# Autodesk Inventor assembly: Pancake Pneumatic Cylinder (217-2778)
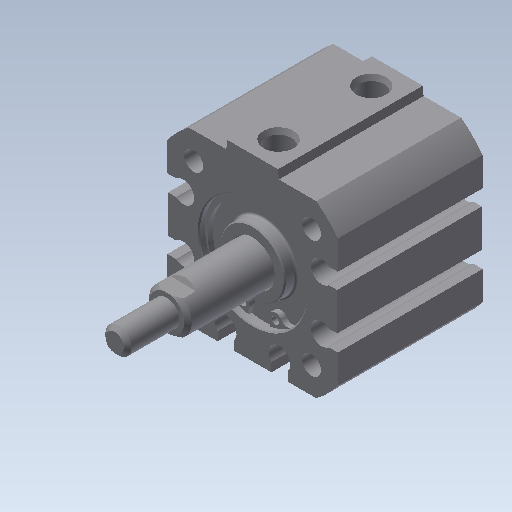
[picture p0: Inventor's stored thumbnail of the model, 512x512]
Saved by Autodesk Inventor 2020 (Build 240168000, 168)
## iProperties
Created: 2014-08-06
Part Number: Pancake Pneumatic Cylinder (217-2778)
Description: STEP AP203
Document SubType Name: Assembly
Designer: mavericks
Sending System: SolidWorks 2014
Preprocessor: SwSTEP 2.0
Title: 217-2778-001 Rev2.STEP
Revision Number: ANY
## Documents named in this file (4)
- T:\EIT\2022 Rapid React\COMMON PARTS\AIR CYLINDERS\Pancake cylinders\Pancake Pneumatic Cylinder (217-2778).iam
- T:\EIT\2022 Rapid React\COMMON PARTS\AIR CYLINDERS\Pancake cylinders\217-2778-NCQ8A075-050M_NCQ8 Tube_075A.ipt
- T:\EIT\2022 Rapid React\COMMON PARTS\AIR CYLINDERS\Pancake cylinders\217-2778-NCQ8A075-050M_NCQ8 Rod_075M.ipt
- T:\EIT\2022 Rapid React\COMMON PARTS\AIR CYLINDERS\Pancake cylinders\217-2778-NCQ8A075-050M_Snap Ring_075.ipt
## Components (3 placed, 3 different names)
1. 217-2778-NCQ8A075-050M_NCQ8 Tube_075A_1 — Mate:1, Mate:2
2. 217-2778-NCQ8A075-050M_NCQ8 Rod_075M_2 — Mate:1, Mate:2
3. 217-2778-NCQ8A075-050M_Snap Ring_075_3
## Relationships (2: Mate 2)
- Mate:1: 217-2778-NCQ8A075-050M_NCQ8 Tube_075A_1 ↔ 217-2778-NCQ8A075-050M_NCQ8 Rod_075M_2
- Mate:2: 217-2778-NCQ8A075-050M_NCQ8 Tube_075A_1 ↔ 217-2778-NCQ8A075-050M_NCQ8 Rod_075M_2
